# Autodesk Inventor assembly: BombaPerisImprimible
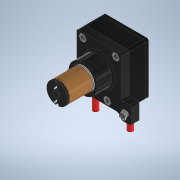
[picture p0: Inventor's stored thumbnail of the model, 180x180]
Saved by Autodesk Inventor 2020.2 (Build 242310000, 310)
## iProperties
Created: 2020-12-04
Part Number: BombaPerisImprimible
Document SubType Name: Assembly
Designer: JK
Sending System: Autodesk Inventor 2020
Preprocessor: ST-DEVELOPER v18
Title: D:\Desk\Drés\2020\Trabajo personal\jk\Podasana\bomba peristaltica\imp\BombaPerisImprimible.stp
Author: andre
## Documents named in this file (13)
- C:\Users\JK\Documents\Inventor\BioMixer\Sist dispensador de líquido viscoso\BombaPeristaltica\BombaPeristaltica.iam
- C:\Users\JK\Documents\Inventor\BioMixer\Sist dispensador de líquido viscoso\BombaPeristaltica\Impulsor.iam
- C:\Users\JK\Documents\Inventor\BioMixer\Sist dispensador de líquido viscoso\BombaPeristaltica\TapaInferior.ipt
- C:\Users\JK\Documents\Inventor\BioMixer\Sist dispensador de líquido viscoso\BombaPeristaltica\TapaSuperior.ipt
- C:\Users\JK\Documents\Inventor\BioMixer\Sist dispensador de líquido viscoso\BombaPeristaltica\PernoM3x6Avellanado.ipt
- C:\Users\JK\Documents\Inventor\BioMixer\Sist dispensador de líquido viscoso\BombaPeristaltica\MotorDC12V100RPM.ipt
- C:\Users\JK\Documents\Inventor\BioMixer\Sist dispensador de líquido viscoso\BombaPeristaltica\GolillaM4DIN125.ipt
- C:\Users\JK\Documents\Inventor\BioMixer\Sist dispensador de líquido viscoso\BombaPeristaltica\Manguera.ipt
- C:\Users\JK\Documents\Inventor\BioMixer\Sist dispensador de líquido viscoso\BombaPeristaltica\CajaBomba.ipt
- C:\Users\JK\Documents\Inventor\BioMixer\Sist dispensador de líquido viscoso\BombaPeristaltica\TuercaM5.ipt
- C:\Users\JK\Documents\Inventor\BioMixer\Sist dispensador de líquido viscoso\BombaPeristaltica\PernoM5x30Plano.ipt
- C:\Users\JK\Documents\Inventor\BioMixer\Sist dispensador de líquido viscoso\BombaPeristaltica\TuercaTM5Perfil2020.ipt
- C:\Users\JK\Documents\Inventor\BioMixer\Sist dispensador de líquido viscoso\BombaPeristaltica\PernoM5x12Plano.ipt
## Components (21 placed, 12 different names)
1. MotorDC12V100RPM:1
2. Impulsor [sub-assembly]
3. Caja — Mate:3, Mate:4, Mate:19, Mate:68, Angle:8, Angle:9, Flush:19
4. TapaSuperior — Mate:3, Mate:4, Flush:19, Mate:83, Mate:84, Mate:85, Mate:86, Mate:87
5. PernoM3x6Avellanado:1 — Flush:10
6. TapaInferior:1 — Mate:19, Flush:12, Angle:8, Mate:82, Mate:88, Angle:10, Mate:92, Mate:93, Mate:94, Mate:95, Mate:98
7. PernoM3x6Avellanado:2 — Flush:10, Flush:12
8. GolillaM4DIN125:1
9. Manguera:1 — Mate:68, Angle:9
10. PernoM5x30Plano:1 — Mate:85, Flush:20, Flush:21
11. PernoM5x30Plano:2 — Mate:86, Flush:22, Mate:90
12. PernoM5x30Plano:3 — Mate:84, Mate:87, Flush:20, Mate:88, Mate:89
13. PernoM5x30Plano:4 — Mate:83, Flush:21, Flush:22, Mate:91
14. TuercaM5:1 — Flush:13, Mate:91, Angle:10, Angle:11, Angle:12
15. TuercaM5:2 — Flush:13, Flush:18, Mate:90, Angle:11
16. TuercaM5:3 — Mate:82, Flush:17, Flush:18, Angle:13
17. TuercaM5:4 — Flush:17, Mate:89, Angle:12, Angle:13, Mate:92
18. TuercaTM5Perfil2020:1 — Mate:96, Angle:14, Mate:98
19. TuercaTM5Perfil2020:2 — Mate:97, Angle:14
20. PernoM5x12Plano:1 — Mate:93, Flush:23, Mate:95, Mate:96
21. PernoM5x12Plano:2 — Mate:94, Flush:23, Mate:97
## Relationships (47: Mate 30, Flush 10, Angle 7)
- Mate:3: Caja ↔ TapaSuperior
- Mate:4: Caja ↔ TapaSuperior
- Mate:19: Caja ↔ TapaInferior:1
- [Mate]: MotorDC12V100RPM:1 ↔ TapaInferior:1
- [Mate]: MotorDC12V100RPM:1 ↔ TapaInferior:1
- [Mate]: MotorDC12V100RPM:1 ↔ PernoM3x6Avellanado:1
- [Mate]: MotorDC12V100RPM:1 ↔ PernoM3x6Avellanado:2
- Flush:10: PernoM3x6Avellanado:1 ↔ PernoM3x6Avellanado:2
- Flush:12: TapaInferior:1 ↔ PernoM3x6Avellanado:2
- [Mate]: MotorDC12V100RPM:1 ↔ TapaInferior:1
- [Mate]: MotorDC12V100RPM:1 ↔ Impulsor
- [Mate]: MotorDC12V100RPM:1 ↔ GolillaM4DIN125:1
- [Mate]: TapaInferior:1 ↔ GolillaM4DIN125:1
- [Mate]: Impulsor ↔ GolillaM4DIN125:1
- Mate:68: Caja ↔ Manguera:1
- Angle:8 (0 deg): Caja ↔ TapaInferior:1
- Angle:9 (0 deg): Caja ↔ Manguera:1
- Flush:13: TuercaM5:1 ↔ TuercaM5:2
- Mate:82: TapaInferior:1 ↔ TuercaM5:3
- Flush:17: TuercaM5:3 ↔ TuercaM5:4
- Flush:18: TuercaM5:2 ↔ TuercaM5:3
- Flush:19: Caja ↔ TapaSuperior
- Mate:83: TapaSuperior ↔ PernoM5x30Plano:4
- Mate:84: TapaSuperior ↔ PernoM5x30Plano:3
- Mate:85: TapaSuperior ↔ PernoM5x30Plano:1
- Mate:86: TapaSuperior ↔ PernoM5x30Plano:2
- Mate:87: TapaSuperior ↔ PernoM5x30Plano:3
- Flush:20: PernoM5x30Plano:1 ↔ PernoM5x30Plano:3
- Flush:21: PernoM5x30Plano:1 ↔ PernoM5x30Plano:4
- Flush:22: PernoM5x30Plano:2 ↔ PernoM5x30Plano:4
- Mate:88: TapaInferior:1 ↔ PernoM5x30Plano:3
- Mate:89: PernoM5x30Plano:3 ↔ TuercaM5:4
- Mate:90: PernoM5x30Plano:2 ↔ TuercaM5:2
- Mate:91: PernoM5x30Plano:4 ↔ TuercaM5:1
- Angle:10 (0 deg): TapaInferior:1 ↔ TuercaM5:1
- Angle:11 (0 deg): TuercaM5:1 ↔ TuercaM5:2
- Angle:12 (0 deg): TuercaM5:1 ↔ TuercaM5:4
- Angle:13 (0 deg): TuercaM5:3 ↔ TuercaM5:4
- Mate:92: TapaInferior:1 ↔ TuercaM5:4
- Mate:93: TapaInferior:1 ↔ PernoM5x12Plano:1
- Mate:94: TapaInferior:1 ↔ PernoM5x12Plano:2
- Flush:23: PernoM5x12Plano:1 ↔ PernoM5x12Plano:2
- Mate:95: TapaInferior:1 ↔ PernoM5x12Plano:1
- Mate:96: TuercaTM5Perfil2020:1 ↔ PernoM5x12Plano:1
- Mate:97: TuercaTM5Perfil2020:2 ↔ PernoM5x12Plano:2
- Angle:14 (0 deg): TuercaTM5Perfil2020:1 ↔ TuercaTM5Perfil2020:2
- Mate:98 (0.8 mm): TapaInferior:1 ↔ TuercaTM5Perfil2020:1
